# Autodesk Inventor assembly: robot arm box
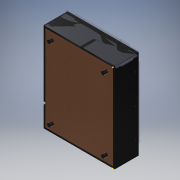
[picture p0: Inventor's stored thumbnail of the model, 180x180]
Saved by Autodesk Inventor 2018 (Build 220112000, 112)
## iProperties
Created: 2017-10-09
Part Number: robot arm box
Document SubType Name: Assembly
Designer: HP
Author: HP
## Documents named in this file (13)
- C:\!_Dani\!_cloud\ownCloud\rover\Robot arm box\robot arm box.iam
- C:\!_Dani\!_cloud\ownCloud\rover\Robot arm box\basic plate.ipt
- C:\!_Dani\!_cloud\ownCloud\rover\Robot arm box\sides.ipt
- C:\!_Dani\!_cloud\ownCloud\rover\Robot arm box\fronts.ipt
- C:\Users\HP\Documents\Inventor\Content Center Files\R2018\en-US\ISO 7046-1 Z(1)\ISO 7046-1 - M3 x 12 - 4.8 - Z - ISO.ipt
- C:\Users\HP\Documents\Inventor\Content Center Files\R2018\en-US\JIS B 1122 - C-Z(2)\JIS B 1122 - ST4,8 x 19 - C - Z(1).ipt
- C:\Users\HP\Documents\Inventor\Content Center Files\R2018\en-US\ISO 4032(2)\ISO 4032 - M3 - ISO.ipt
- C:\!_Dani\!_cloud\ownCloud\rover\Robot arm box\top.ipt
- C:\!_Dani\!_cloud\ownCloud\rover\Robot arm box\Dávidtól fedlap\Part1^package.ipt
- C:\!_Dani\!_cloud\ownCloud\rover\Robot arm box\Dávidtól fedlap\Part3^package.ipt
- C:\!_Dani\!_cloud\ownCloud\rover\Robot arm box\sides\sides-01.ipt
- C:\!_Dani\!_cloud\ownCloud\rover\Robot arm box\Dávidtól fedlap\Part6^package.ipt
- C:\!_Dani\!_cloud\ownCloud\rover\Robot arm box\robot arm box parameters.xlsx
## Components (12 placed, 11 different names)
1. basic plate:1 — Flush:2, Mate:1, Mate:2, Flush:3, Flush:5, Mate:3, Flush:10, Flush:13
2. Part3^package:1 — Mate:19, Mate:20, Mate:21
3. sides-01:3 — Flush:3, Flush:6, Mate:19, Mate:20, Mate:21
4. sides:2 — Flush:5, Flush:6, Mate:3, Flush:9, Flush:12, Mate:16, Mate:18
5. Part6^package:1 — Flush:23, Mate:22, Mate:23
6. fronts:1 — Flush:9, Flush:11, Flush:13
7. fronts:2 — Flush:10, Flush:11, Flush:12, Flush:23, Mate:23
8. ISO 7046-1 Z M3 x 12 - 4.8 - Z:1
9. JIS B 1122 - C-Z ST4,8 x 19 - C - Z:1
10. ISO 4032 M3:1
11. Part1^package:1 — Mate:4, Mate:16, Mate:17, Mate:18
12. top:1 — Mate:4, Mate:17, Mate:22
## Relationships (22: Mate 12, Flush 10)
- Flush:2: basic plate:1
- Mate:1: basic plate:1
- Mate:2: basic plate:1
- Flush:3: basic plate:1 ↔ sides-01:3
- Flush:5: basic plate:1 ↔ sides:2
- Flush:6: sides-01:3 ↔ sides:2
- Mate:3: basic plate:1 ↔ sides:2
- Flush:9: sides:2 ↔ fronts:1
- Flush:10: basic plate:1 ↔ fronts:2
- Flush:11: fronts:1 ↔ fronts:2
- Flush:12: sides:2 ↔ fronts:2
- Flush:13: basic plate:1 ↔ fronts:1
- Mate:4: Part1^package:1 ↔ top:1
- Mate:16: sides:2 ↔ Part1^package:1
- Mate:17: Part1^package:1 ↔ top:1
- Mate:18: sides:2 ↔ Part1^package:1
- Mate:19: Part3^package:1 ↔ sides-01:3
- Mate:20: Part3^package:1 ↔ sides-01:3
- Mate:21: Part3^package:1 ↔ sides-01:3
- Flush:23: Part6^package:1 ↔ fronts:2
- Mate:22: Part6^package:1 ↔ top:1
- Mate:23: Part6^package:1 ↔ fronts:2
## Named parameters: plate_thickness = 5 mm, ABS_tolerance = 0 mm, laser_cutter_thickness = 0.1 mm, basic_plate_offset = 0 mm
